# Autodesk Inventor assembly: pendulum_assembly
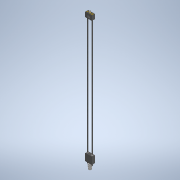
[picture p0: Inventor's stored thumbnail of the model, 180x180]
Saved by Autodesk Inventor 2021 (Build 250183000, 183)
## iProperties
Created: 2022-07-01
Part Number: pendulum_assembly
Document SubType Name: Assembly
Designer: lenna
Author: lenna
## Documents named in this file (10)
- C:\Users\lenna\Desktop\Lennart\Uni\Master\2. Semester\SDM\CAD_neu\pendulum_assembly.iam
- C:\Users\lenna\Desktop\Lennart\Uni\Master\2. Semester\SDM\CAD_neu\pendulum_adapter.ipt
- C:\Users\lenna\Desktop\Lennart\Uni\Master\2. Semester\SDM\CAD_neu\M3_threaded_rod_460.ipt
- C:\Users\lenna\Desktop\Lennart\Uni\Master\2. Semester\SDM\CAD_neu\M3_tread_insert.ipt
- C:\Users\lenna\Desktop\Lennart\Uni\Master\2. Semester\SDM\CAD_neu\pendulum_mass.ipt
- C:\Users\lenna\Desktop\Lennart\Uni\Master\2. Semester\SDM\CAD_neu\clamping_insert.ipt
- C:\Users\lenna\Documents\Inventor\Content Center Files\R2021\en-US\DIN EN ISO 4035\DIN EN ISO 4035 - M3.ipt
- C:\Users\lenna\Documents\Inventor\Content Center Files\R2021\en-US\ISO 4762(1)\DIN EN ISO 4762 - M3 x 10.ipt
- C:\Users\lenna\Documents\Inventor\Content Center Files\R2021\en-US\ISO 4762(1)\DIN EN ISO 4762 - M6 x 30.ipt
- C:\Users\lenna\Documents\Inventor\Content Center Files\R2021\en-US\DIN EN ISO 4032\DIN EN ISO 4032 - M6.ipt
## Components (16 placed, 9 different names)
1. pendulum_adapter:1 — Insert:1, Insert:2
2. M3_tread_insert:2 — Insert:2, Insert:7
3. pendulum_mass:1 — Mate:1, Insert:4, Insert:5, Insert:6, Mate:2
4. clamping_insert:1 — Insert:4, Insert:8
5. DIN EN ISO 4762 M3 x 10:1 — Insert:7
6. DIN EN ISO 4762 M6 x 30:1 — Insert:8, Insert:10
7. DIN EN ISO 4032 M6:1 — Insert:9, Insert:10
8. DIN EN ISO 4032 M6:2 — Insert:9
9. M3_tread_insert:1 — Insert:1, Insert:3
10. M3_threaded_rod_460:1 — Insert:3, Mate:1, Flush:1
11. DIN EN ISO 4035 M3:2 — Insert:6
12. DIN EN ISO 4035 M3:1 — Insert:5, Flush:1
13. M3_tread_insert:3
14. M3_threaded_rod_460:2 — Mate:2
15. DIN EN ISO 4035 M3:3
16. DIN EN ISO 4035 M3:4
## Component patterns: (2 elements, first: M3_tread_insert:1 + M3_threaded_rod_460:1 + DIN EN ISO 4035 M3:2 + DIN EN ISO 4035 M3:1)
## Relationships (13: Insert 10, Mate 2, Flush 1)
- Insert:1: pendulum_adapter:1 ↔ M3_tread_insert:1
- Insert:2: pendulum_adapter:1 ↔ M3_tread_insert:2
- Insert:3: M3_tread_insert:1 ↔ M3_threaded_rod_460:1
- Mate:1: pendulum_mass:1 ↔ M3_threaded_rod_460:1
- Insert:4: pendulum_mass:1 ↔ clamping_insert:1
- Insert:5: pendulum_mass:1 ↔ DIN EN ISO 4035 M3:1
- Insert:6: pendulum_mass:1 ↔ DIN EN ISO 4035 M3:2
- Mate:2: pendulum_mass:1 ↔ M3_threaded_rod_460:2
- Flush:1 (5 mm): M3_threaded_rod_460:1 ↔ DIN EN ISO 4035 M3:1
- Insert:7 (2.5 mm): M3_tread_insert:2 ↔ DIN EN ISO 4762 M3 x 10:1
- Insert:8 (15 mm): clamping_insert:1 ↔ DIN EN ISO 4762 M6 x 30:1
- Insert:9: DIN EN ISO 4032 M6:1 ↔ DIN EN ISO 4032 M6:2
- Insert:10 (2 mm): DIN EN ISO 4762 M6 x 30:1 ↔ DIN EN ISO 4032 M6:1
